# Autodesk Inventor assembly: КВ33.044.500 - Каретка оси Y
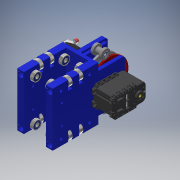
[picture p0: Inventor's stored thumbnail of the model, 180x180]
Saved by Autodesk Inventor 2019 (Build 230136000, 136)
## iProperties
Created: 2019-07-21
Part Number: КВ33.044.500 - Каретка оси Y
Material: Типовые
Document SubType Name: Assembly
Designer: Петров Иван
Author: Петров Иван
## Documents named in this file (11)
- E:\IVAN\Kvantoriada2019\optimal_gripper\hardware\КВ33.044.600 - Каретка оси Y.iam
- E:\IVAN\Kvantoriada2019\optimal_gripper\hardware\КВ33.044.601 - Щека каретка оси Y.ipt
- E:\IVAN\Kvantoriada2019\optimal_gripper\hardware\Стандартные изделия\Подшипник 624Z.ipt
- E:\IVAN\Kvantoriada2019\optimal_gripper\hardware\Стандартные изделия\Сервомотор Dynamixel AX-12A\ax-12a.iam
- E:\IVAN\Kvantoriada2019\optimal_gripper\hardware\Стандартные изделия\Колесо оптического датчика.ipt
- E:\IVAN\Kvantoriada2019\optimal_gripper\hardware\Стандартные изделия\Шкив большой Makeblock.ipt
- E:\IVAN\Kvantoriada2019\optimal_gripper\hardware\Стандартные изделия\Боковина шкива.ipt
- E:\IVAN\Kvantoriada2019\optimal_gripper\hardware\Стандартные изделия\Датчик оптический стандартный.ipt
- E:\IVAN\Kvantoriada2019\optimal_gripper\hardware\Стандартные изделия\Проставка 6.5 мм.ipt
- E:\IVAN\Kvantoriada2019\optimal_gripper\hardware\КВ33.044.800 - Шкив плоский Makeblock сборка.iam
- E:\IVAN\Kvantoriada2019\optimal_gripper\hardware\Стандартные изделия\Концевик механический\Концевик механический.ipt
## Components (27 placed, 10 different names)
1. КВ33.044.601 - Щека каретка оси Y:1 — Совмещение:1, Совмещение:2, Совмещение:3, Совмещение:4, Совмещение:5, Совмещение:6, 2.5, Совмещение:8, Совмещение:9, Совмещение:10, Совмещение:11, Совмещение:12, Совмещение:13, Совмещение:14, Совмещение:15, Совмещение:16, Совмещение:23, Совмещение:24, Совмещение:25, Совмещение:26, Совмещение:27, Совмещение:28, Совмещение:29, Совмещение:30, Совмещение:31, Совмещение:32, Совмещение:33, Совмещение:34, Совмещение:35, Совмещение:36, Совмещение:37, Совмещение:38, Совмещение:40, Совмещение:41, Совмещение:53, Совмещение:54, Совмещение:55, Совмещение:56, Касательность:1, Касательность:2, Совмещение:57, Совмещение:58, Совмещение:59, Совмещение:60, Угол:1, Совмещение:61, Совмещение:62, Угол:2
2. Подшипник 624Z:1 — Совмещение:1, Совмещение:8
3. Подшипник 624Z:2 — Совмещение:4, Совмещение:5
4. Подшипник 624Z:3 — Совмещение:3, Совмещение:6
5. Подшипник 624Z:4 — Совмещение:2, 2.5
6. Подшипник 624Z:5 — Совмещение:9, Совмещение:15
7. Подшипник 624Z:6 — Совмещение:10, Совмещение:16
8. Подшипник 624Z:7 — Совмещение:11, Совмещение:13
9. Подшипник 624Z:8 — Совмещение:12, Совмещение:14
10. Подшипник 624Z:9 — Совмещение:23, Совмещение:24
11. Подшипник 624Z:10 — Совмещение:25, Совмещение:26
12. Подшипник 624Z:11 — Совмещение:27, Совмещение:28
13. Подшипник 624Z:12 — Совмещение:29, Совмещение:30
14. Подшипник 624Z:13 — Совмещение:31, Совмещение:32
15. Подшипник 624Z:14 — Совмещение:33, Совмещение:34
16. Подшипник 624Z:15 — Совмещение:35, Совмещение:36
17. Подшипник 624Z:16 — Совмещение:37, Совмещение:38
18. ax-12a:1 [sub-assembly] — Совмещение:40, Совмещение:41, Совмещение:42, Совмещение:43, Совмещение:58
19. Проставка 6.5 мм:1 — Совмещение:42, Совмещение:43, Совмещение:44, Совмещение:45, Совмещение:46
20. Колесо оптического датчика:1 — Совмещение:44, Совмещение:45, Совмещение:46, Совмещение:47, Совмещение:48, Совмещение:49
21. Шкив большой Makeblock:1 — Совмещение:47, Совмещение:48, Совмещение:49, Совмещение:50, Совмещение:51, Совмещение:52
22. Боковина шкива:1 — Совмещение:50, Совмещение:51, Совмещение:52
23. Датчик оптический стандартный:1 — Совмещение:53, Совмещение:54, Совмещение:55
24. КВ33.044.800 - Шкив плоский Makeblock сборка:1 [sub-assembly] — Совмещение:56, Касательность:1
25. КВ33.044.800 - Шкив плоский Makeblock сборка:2 [sub-assembly] — Касательность:2, Совмещение:57
26. Концевик механический:1 — Совмещение:59, Совмещение:60, Угол:1
27. Концевик механический:2 — Совмещение:61, Совмещение:62, Угол:2
## Relationships (59: Mate 55, Tangent 2, Angle 2)
- Совмещение:1 [Mate]: КВ33.044.601 - Щека каретка оси Y:1 ↔ Подшипник 624Z:1
- Совмещение:2 [Mate]: КВ33.044.601 - Щека каретка оси Y:1 ↔ Подшипник 624Z:4
- Совмещение:3 [Mate]: КВ33.044.601 - Щека каретка оси Y:1 ↔ Подшипник 624Z:3
- Совмещение:4 [Mate]: КВ33.044.601 - Щека каретка оси Y:1 ↔ Подшипник 624Z:2
- Совмещение:5 [Mate] (2.5 mm): КВ33.044.601 - Щека каретка оси Y:1 ↔ Подшипник 624Z:2
- Совмещение:6 [Mate] (2.5 mm): КВ33.044.601 - Щека каретка оси Y:1 ↔ Подшипник 624Z:3
- 2.5 [Mate] (2.5 mm): КВ33.044.601 - Щека каретка оси Y:1 ↔ Подшипник 624Z:4
- Совмещение:8 [Mate] (2.5 mm): КВ33.044.601 - Щека каретка оси Y:1 ↔ Подшипник 624Z:1
- Совмещение:9 [Mate]: КВ33.044.601 - Щека каретка оси Y:1 ↔ Подшипник 624Z:5
- Совмещение:10 [Mate]: КВ33.044.601 - Щека каретка оси Y:1 ↔ Подшипник 624Z:6
- Совмещение:11 [Mate]: КВ33.044.601 - Щека каретка оси Y:1 ↔ Подшипник 624Z:7
- Совмещение:12 [Mate]: КВ33.044.601 - Щека каретка оси Y:1 ↔ Подшипник 624Z:8
- Совмещение:13 [Mate] (0.5 mm): КВ33.044.601 - Щека каретка оси Y:1 ↔ Подшипник 624Z:7
- Совмещение:14 [Mate] (0.5 mm): КВ33.044.601 - Щека каретка оси Y:1 ↔ Подшипник 624Z:8
- Совмещение:15 [Mate] (0.5 mm): КВ33.044.601 - Щека каретка оси Y:1 ↔ Подшипник 624Z:5
- Совмещение:16 [Mate] (0.5 mm): КВ33.044.601 - Щека каретка оси Y:1 ↔ Подшипник 624Z:6
- Совмещение:23 [Mate]: КВ33.044.601 - Щека каретка оси Y:1 ↔ Подшипник 624Z:9
- Совмещение:24 [Mate] (0.5 mm): КВ33.044.601 - Щека каретка оси Y:1 ↔ Подшипник 624Z:9
- Совмещение:25 [Mate]: КВ33.044.601 - Щека каретка оси Y:1 ↔ Подшипник 624Z:10
- Совмещение:26 [Mate] (0.5 mm): КВ33.044.601 - Щека каретка оси Y:1 ↔ Подшипник 624Z:10
- Совмещение:27 [Mate]: КВ33.044.601 - Щека каретка оси Y:1 ↔ Подшипник 624Z:11
- Совмещение:28 [Mate] (0.5 mm): КВ33.044.601 - Щека каретка оси Y:1 ↔ Подшипник 624Z:11
- Совмещение:29 [Mate]: КВ33.044.601 - Щека каретка оси Y:1 ↔ Подшипник 624Z:12
- Совмещение:30 [Mate] (0.5 mm): КВ33.044.601 - Щека каретка оси Y:1 ↔ Подшипник 624Z:12
- Совмещение:31 [Mate]: КВ33.044.601 - Щека каретка оси Y:1 ↔ Подшипник 624Z:13
- Совмещение:32 [Mate] (2.5 mm): КВ33.044.601 - Щека каретка оси Y:1 ↔ Подшипник 624Z:13
- Совмещение:33 [Mate]: КВ33.044.601 - Щека каретка оси Y:1 ↔ Подшипник 624Z:14
- Совмещение:34 [Mate] (2.5 mm): КВ33.044.601 - Щека каретка оси Y:1 ↔ Подшипник 624Z:14
- Совмещение:35 [Mate] (2.5 mm): КВ33.044.601 - Щека каретка оси Y:1 ↔ Подшипник 624Z:15
- Совмещение:36 [Mate]: КВ33.044.601 - Щека каретка оси Y:1 ↔ Подшипник 624Z:15
- Совмещение:37 [Mate] (2.5 mm): КВ33.044.601 - Щека каретка оси Y:1 ↔ Подшипник 624Z:16
- Совмещение:38 [Mate]: КВ33.044.601 - Щека каретка оси Y:1 ↔ Подшипник 624Z:16
- Совмещение:40 [Mate]: КВ33.044.601 - Щека каретка оси Y:1 ↔ ax-12a:1
- Совмещение:41 [Mate]: КВ33.044.601 - Щека каретка оси Y:1 ↔ ax-12a:1
- Совмещение:42 [Mate]: ax-12a:1 ↔ Проставка 6.5 мм:1
- Совмещение:43 [Mate]: ax-12a:1 ↔ Проставка 6.5 мм:1
- Совмещение:44 [Mate]: Проставка 6.5 мм:1 ↔ Колесо оптического датчика:1
- Совмещение:45 [Mate]: Проставка 6.5 мм:1 ↔ Колесо оптического датчика:1
- Совмещение:46 [Mate]: Проставка 6.5 мм:1 ↔ Колесо оптического датчика:1
- Совмещение:47 [Mate]: Колесо оптического датчика:1 ↔ Шкив большой Makeblock:1
- Совмещение:48 [Mate]: Колесо оптического датчика:1 ↔ Шкив большой Makeblock:1
- Совмещение:49 [Mate]: Колесо оптического датчика:1 ↔ Шкив большой Makeblock:1
- Совмещение:50 [Mate]: Шкив большой Makeblock:1 ↔ Боковина шкива:1
- Совмещение:51 [Mate]: Шкив большой Makeblock:1 ↔ Боковина шкива:1
- Совмещение:52 [Mate]: Шкив большой Makeblock:1 ↔ Боковина шкива:1
- Совмещение:53 [Mate]: КВ33.044.601 - Щека каретка оси Y:1 ↔ Датчик оптический стандартный:1
- Совмещение:54 [Mate]: КВ33.044.601 - Щека каретка оси Y:1 ↔ Датчик оптический стандартный:1
- Совмещение:55 [Mate]: КВ33.044.601 - Щека каретка оси Y:1 ↔ Датчик оптический стандартный:1
- Совмещение:56 [Mate]: КВ33.044.601 - Щека каретка оси Y:1 ↔ КВ33.044.800 - Шкив плоский Makeblock сборка:1
- Касательность:1 [Tangent]: КВ33.044.601 - Щека каретка оси Y:1 ↔ КВ33.044.800 - Шкив плоский Makeblock сборка:1
- Касательность:2 [Tangent]: КВ33.044.601 - Щека каретка оси Y:1 ↔ КВ33.044.800 - Шкив плоский Makeblock сборка:2
- Совмещение:57 [Mate]: КВ33.044.601 - Щека каретка оси Y:1 ↔ КВ33.044.800 - Шкив плоский Makeblock сборка:2
- Совмещение:58 [Mate]: КВ33.044.601 - Щека каретка оси Y:1 ↔ ax-12a:1
- Совмещение:59 [Mate]: КВ33.044.601 - Щека каретка оси Y:1 ↔ Концевик механический:1
- Совмещение:60 [Mate]: КВ33.044.601 - Щека каретка оси Y:1 ↔ Концевик механический:1
- Угол:1 [Angle] (0 deg): КВ33.044.601 - Щека каретка оси Y:1 ↔ Концевик механический:1
- Совмещение:61 [Mate]: КВ33.044.601 - Щека каретка оси Y:1 ↔ Концевик механический:2
- Совмещение:62 [Mate]: КВ33.044.601 - Щека каретка оси Y:1 ↔ Концевик механический:2
- Угол:2 [Angle] (0 deg): КВ33.044.601 - Щека каретка оси Y:1 ↔ Концевик механический:2
